# Autodesk Inventor assembly: Tracker Wheel Right
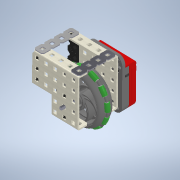
[picture p0: Inventor's stored thumbnail of the model, 180x180]
Saved by Autodesk Inventor 2020 (Build 240168000, 168)
## iProperties
Created: 2019-09-01
Part Number: Tracker Wheel Right
Document SubType Name: Assembly
Designer: Corey
Author: Corey
## Documents named in this file (7)
- D:\Robotics\20192020 Tower Takeover\CAD\Tracker Wheel Right.iam
- D:\Robotics\20192020 Tower Takeover\CAD\Parts\Motion\Wheels & Rollers\2.75'' Omni-Directional Wheel_MIR.iam
- D:\Robotics\20192020 Tower Takeover\CAD\Parts\Motion\Bearing Flat_MIR2.ipt
- D:\Robotics\20192020 Tower Takeover\CAD\Parts\Motion\Drive Shafts\Drive Shaft 3''_MIR1.ipt
- D:\Robotics\20192020 Tower Takeover\CAD\Parts\Electronics\Optical Shaft Encoder_MIR2.iam
- D:\Robotics\20192020 Tower Takeover\CAD\Parts\Structure\C-Channels\Aluminum\5-Wide\Aluminum C-Channel 1x5x1x5_MIR2.ipt
- D:\Robotics\20192020 Tower Takeover\CAD\Parts\Structure\1 Wide Bar\Bar 1x4_MIR2.ipt
## Components (10 placed, 6 different names)
1. 2.75'' Omni-Directional Wheel_MIR:1 [sub-assembly] — Flush:28, Mate:24, Mate:25
2. Bearing Flat_MIR2:1 — Insert:8, Insert:9, Insert:10
3. Drive Shaft 3''_MIR1:1 — Insert:8, Flush:28, Mate:24, Mate:25
4. Optical Shaft Encoder_MIR2:1 [sub-assembly] — Mate:26, Flush:29, Mate:27
5. Aluminum C-Channel 1x5x1x5_MIR2:1 — Mate:26, Flush:29, Mate:27, Insert:13, Insert:14, Mate:28, Flush:32, Flush:33, Mate:29
6. Aluminum C-Channel 1x5x1x5_MIR2:2 — Insert:9, Insert:10, Insert:11, Insert:12, Flush:30, Flush:31, Flush:34, Flush:35, Mate:30
7. Bearing Flat_MIR2:2 — Insert:11, Insert:12
8. Bearing Flat_MIR2:3 — Insert:13, Insert:14
9. Bar 1x4_MIR2:1 — Mate:28, Flush:30, Flush:31
10. Bar 1x4_MIR2:2 — Flush:32, Flush:33, Mate:29, Flush:34, Flush:35, Mate:30
## Relationships (22: Flush 8, Insert 7, Mate 7)
- Insert:8 (-6.35 mm): Bearing Flat_MIR2:1 ↔ Drive Shaft 3''_MIR1:1
- Flush:28 (22.098 mm): 2.75'' Omni-Directional Wheel_MIR:1 ↔ Drive Shaft 3''_MIR1:1
- Mate:24: 2.75'' Omni-Directional Wheel_MIR:1 ↔ Drive Shaft 3''_MIR1:1
- Mate:25: 2.75'' Omni-Directional Wheel_MIR:1 ↔ Drive Shaft 3''_MIR1:1
- Mate:26 (1.016 mm): Optical Shaft Encoder_MIR2:1 ↔ Aluminum C-Channel 1x5x1x5_MIR2:1
- Flush:29: Optical Shaft Encoder_MIR2:1 ↔ Aluminum C-Channel 1x5x1x5_MIR2:1
- Mate:27: Optical Shaft Encoder_MIR2:1 ↔ Aluminum C-Channel 1x5x1x5_MIR2:1
- Insert:9: Bearing Flat_MIR2:1 ↔ Aluminum C-Channel 1x5x1x5_MIR2:2
- Insert:10: Bearing Flat_MIR2:1 ↔ Aluminum C-Channel 1x5x1x5_MIR2:2
- Insert:11: Aluminum C-Channel 1x5x1x5_MIR2:2 ↔ Bearing Flat_MIR2:2
- Insert:12: Aluminum C-Channel 1x5x1x5_MIR2:2 ↔ Bearing Flat_MIR2:2
- Insert:13: Aluminum C-Channel 1x5x1x5_MIR2:1 ↔ Bearing Flat_MIR2:3
- Insert:14: Aluminum C-Channel 1x5x1x5_MIR2:1 ↔ Bearing Flat_MIR2:3
- Mate:28: Aluminum C-Channel 1x5x1x5_MIR2:1 ↔ Bar 1x4_MIR2:1
- Flush:30: Aluminum C-Channel 1x5x1x5_MIR2:2 ↔ Bar 1x4_MIR2:1
- Flush:31: Aluminum C-Channel 1x5x1x5_MIR2:2 ↔ Bar 1x4_MIR2:1
- Flush:32: Aluminum C-Channel 1x5x1x5_MIR2:1 ↔ Bar 1x4_MIR2:2
- Flush:33: Aluminum C-Channel 1x5x1x5_MIR2:1 ↔ Bar 1x4_MIR2:2
- Mate:29: Aluminum C-Channel 1x5x1x5_MIR2:1 ↔ Bar 1x4_MIR2:2
- Flush:34: Aluminum C-Channel 1x5x1x5_MIR2:2 ↔ Bar 1x4_MIR2:2
- Flush:35: Aluminum C-Channel 1x5x1x5_MIR2:2 ↔ Bar 1x4_MIR2:2
- Mate:30: Aluminum C-Channel 1x5x1x5_MIR2:2 ↔ Bar 1x4_MIR2:2
